# Autodesk Inventor assembly: A_Aft
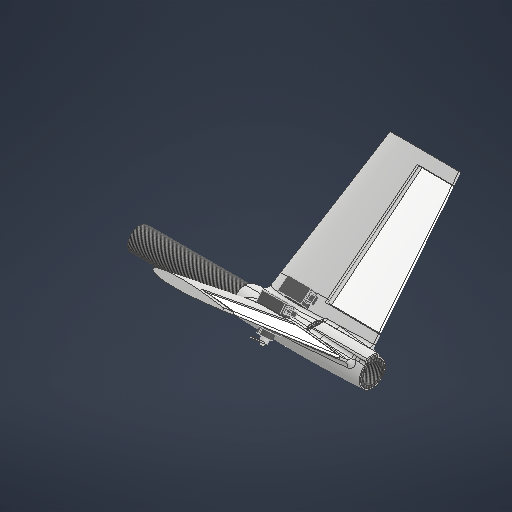
[picture p0: Inventor's stored thumbnail of the model, 512x512]
Saved by Autodesk Inventor 2026 (Build 300175000, 175)
## iProperties
Created: 2025-09-10
Part Number: A_Aft
Document SubType Name: Assembly
Designer: FAL
Author: FAL
## Documents named in this file (16)
- C:\Users\FAL\Projekte\Git\AIRBERT\CAD\Aft\A_Aft.iam
- C:\Users\FAL\Projekte\Git\AIRBERT\CAD\Aft\P_aft_V.ipt
- C:\Users\FAL\Projekte\Git\AIRBERT\CAD\Aft\P_aft_V_rudder.ipt
- C:\Users\FAL\Projekte\Git\AIRBERT\CAD\Aft\P_Carbon_Pipe_Back.ipt
- C:\Users\FAL\Projekte\Git\AIRBERT\CAD\Electronic\P_Servo_27x12.ipt
- C:\Users\FAL\Projekte\Git\AIRBERT\CAD\Aft\P_Aft_body_pipe_connector_inlet_movable.ipt
- C:\Users\FAL\Projekte\Git\AIRBERT\CAD\Aft\P_aft_body_pipe_connector_nut.ipt
- C:\Users\FAL\Projekte\Git\AIRBERT\CAD\Aft\mirror\P_aft_V_rudder_MIR1.ipt
- C:\Users\FAL\Projekte\Git\AIRBERT\CAD\Aft\P_aft_V_wing.ipt
- C:\Users\FAL\Projekte\Git\AIRBERT\CAD\Aft\P_aft_V_body.ipt
- C:\Users\FAL\Projekte\Git\AIRBERT\CAD\Aft\mirror\P_aft_V_wing_MIR.ipt
- C:\Users\FAL\Projekte\Git\AIRBERT\CAD\Electronic\P_Servo_SIMPROP_lever.ipt
- C:\Users\FAL\Projekte\Git\AIRBERT\CAD\Aft\P_aft_servolink.ipt
- C:\Users\FAL\Projekte\Git\AIRBERT\CAD\Electronic\P_Servo_SIMPROP_ex.ipt
- C:\Users\FAL\Projekte\Git\AIRBERT\CAD\Aft\P_aft_Harnes.ipt
- C:\Users\FAL\Projekte\Git\AIRBERT\CAD\Aft\P_aft_V_cap.ipt
## Components (17 placed, 15 different names)
1. P_aft_V:1 — Passend:12, Fluchtend:20, Fluchtend:21, Fluchtend:22, Fluchtend:23, Fluchtend:24
2. P_aft_V_rudder:1 — Fluchtend:22, Fluchtend:23, Fluchtend:24, Passend:26, Passend:38, Passend:49
3. P_Carbon_Pipe_Back:1 — Passend:11, Fluchtend:19, Passend:12, Fluchtend:21, Fluchtend:42
4. P_Servo_27x12:1 — Passend:22, Passend:23, Passend:59, Passend:63, Passend:64
5. P_Servo_27x12:2 — Passend:21, Passend:24, Passend:60, Passend:61, Passend:62
6. P_Aft_body_pipe_connector_inlet_movable:1 — Fluchtend:16, Fluchtend:17, Fluchtend:18, Fluchtend:19
7. P_aft_body_pipe_connector_nut:1 — Fluchtend:13, Fluchtend:14, Fluchtend:15
8. P_aft_V_rudder_MIR1:1 — Passend:30, Passend:31, Passend:39, Passend:44
9. P_aft_V_wing:1 — Fluchtend:26, Fluchtend:27, Fluchtend:31, Passend:38, Passend:49, Passend:64
10. P_aft_V_body:1 — Fluchtend:29, Fluchtend:30, Fluchtend:31, Fluchtend:36, Fluchtend:37, Fluchtend:41, Passend:44, Fluchtend:42, Passend:59, Passend:60, Passend:61, Passend:62, Passend:63
11. P_aft_V_wing_MIR:1 — Passend:19, Passend:20, Fluchtend:36, Passend:30, Passend:31, Passend:39
12. P_Servo_SIMPROP_lever:1 — Passend:21, Passend:24
13. P_Servo_SIMPROP_lever:2 — Passend:22, Passend:23, Passend:25
14. P_aft_servolink:1 — Passend:25, Passend:27, Passend:28
15. P_Servo_SIMPROP_ex:1 — Passend:26, Passend:27, Passend:28
16. P_aft_Harnes:1 — Fluchtend:33, Fluchtend:34, Fluchtend:35
17. P_aft_V_cap:1 — Fluchtend:39, Fluchtend:40, Fluchtend:41
## Relationships (50: Flush 26, Mate 24)
- Fluchtend:13 [Flush]: P_aft_body_pipe_connector_nut:1
- Fluchtend:14 [Flush]: P_aft_body_pipe_connector_nut:1
- Fluchtend:15 [Flush]: P_aft_body_pipe_connector_nut:1
- Passend:11 [Mate]: P_Carbon_Pipe_Back:1
- Fluchtend:16 [Flush]: P_Aft_body_pipe_connector_inlet_movable:1
- Fluchtend:17 [Flush]: P_Aft_body_pipe_connector_inlet_movable:1
- Fluchtend:18 [Flush]: P_Aft_body_pipe_connector_inlet_movable:1
- Fluchtend:19 [Flush]: P_Carbon_Pipe_Back:1 ↔ P_Aft_body_pipe_connector_inlet_movable:1
- Passend:12 [Mate]: P_aft_V:1 ↔ P_Carbon_Pipe_Back:1
- Fluchtend:20 [Flush]: P_aft_V:1
- Fluchtend:21 [Flush]: P_aft_V:1 ↔ P_Carbon_Pipe_Back:1
- Fluchtend:22 [Flush]: P_aft_V:1 ↔ P_aft_V_rudder:1
- Fluchtend:23 [Flush]: P_aft_V:1 ↔ P_aft_V_rudder:1
- Fluchtend:24 [Flush]: P_aft_V:1 ↔ P_aft_V_rudder:1
- Fluchtend:26 [Flush]: P_aft_V_wing:1
- Fluchtend:27 [Flush]: P_aft_V_wing:1
- Fluchtend:29 [Flush]: P_aft_V_body:1
- Fluchtend:30 [Flush]: P_aft_V_body:1
- Fluchtend:31 [Flush]: P_aft_V_wing:1 ↔ P_aft_V_body:1
- Passend:19 [Mate]: P_aft_V_wing_MIR:1
- Passend:20 [Mate]: P_aft_V_wing_MIR:1
- Passend:21 [Mate]: P_Servo_27x12:2 ↔ P_Servo_SIMPROP_lever:1
- Passend:22 [Mate]: P_Servo_27x12:1 ↔ P_Servo_SIMPROP_lever:2
- Passend:23 [Mate]: P_Servo_27x12:1 ↔ P_Servo_SIMPROP_lever:2
- Passend:24 [Mate]: P_Servo_27x12:2 ↔ P_Servo_SIMPROP_lever:1
- Passend:25 [Mate]: P_Servo_SIMPROP_lever:2 ↔ P_aft_servolink:1
- Passend:26 [Mate]: P_aft_V_rudder:1 ↔ P_Servo_SIMPROP_ex:1
- Passend:27 [Mate]: P_aft_servolink:1 ↔ P_Servo_SIMPROP_ex:1
- Passend:28 [Mate] (-15 mm): P_aft_servolink:1 ↔ P_Servo_SIMPROP_ex:1
- Fluchtend:33 [Flush]: P_aft_Harnes:1
- Fluchtend:34 [Flush]: P_aft_Harnes:1
- Fluchtend:35 [Flush]: P_aft_Harnes:1
- Fluchtend:36 [Flush]: P_aft_V_body:1 ↔ P_aft_V_wing_MIR:1
- Passend:30 [Mate]: P_aft_V_rudder_MIR1:1 ↔ P_aft_V_wing_MIR:1
- Passend:31 [Mate]: P_aft_V_rudder_MIR1:1 ↔ P_aft_V_wing_MIR:1
- Fluchtend:37 [Flush]: P_aft_V_body:1
- Passend:38 [Mate]: P_aft_V_rudder:1 ↔ P_aft_V_wing:1
- Passend:39 [Mate]: P_aft_V_rudder_MIR1:1 ↔ P_aft_V_wing_MIR:1
- Fluchtend:39 [Flush]: P_aft_V_cap:1
- Fluchtend:40 [Flush]: P_aft_V_cap:1
- Fluchtend:41 [Flush]: P_aft_V_body:1 ↔ P_aft_V_cap:1
- Passend:44 [Mate]: P_aft_V_rudder_MIR1:1 ↔ P_aft_V_body:1
- Fluchtend:42 [Flush]: P_Carbon_Pipe_Back:1 ↔ P_aft_V_body:1
- Passend:49 [Mate]: P_aft_V_rudder:1 ↔ P_aft_V_wing:1
- Passend:59 [Mate]: P_Servo_27x12:1 ↔ P_aft_V_body:1
- Passend:60 [Mate]: P_Servo_27x12:2 ↔ P_aft_V_body:1
- Passend:61 [Mate]: P_Servo_27x12:2 ↔ P_aft_V_body:1
- Passend:62 [Mate]: P_Servo_27x12:2 ↔ P_aft_V_body:1
- Passend:63 [Mate]: P_Servo_27x12:1 ↔ P_aft_V_body:1
- Passend:64 [Mate]: P_Servo_27x12:1 ↔ P_aft_V_wing:1
